# Autodesk Inventor assembly: RealSense
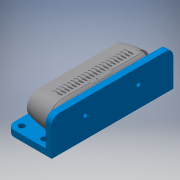
[picture p0: Inventor's stored thumbnail of the model, 180x180]
Saved by Autodesk Inventor 2019 (Build 230136000, 136)
## iProperties
Created: 2020-03-14
Part Number: RealSense
Document SubType Name: Assembly
Designer: james
Author: james
## Documents named in this file (3)
- F:\JimsRobot\FIRSTRobots\Design\Library\Jims\RealSense.iam
- F:\JimsRobot\FIRSTRobots\Design\Library\Jims\Realsense.ipt
- F:\JimsRobot\FIRSTRobots\Design\Library\Intel\000_TA_DS5_DEV_KIT_AWG_RGB_ASM__ASM.iam
## Components (2 placed, 2 different names)
1. Realsense:1 — Mate:1, Mate:2
2. 000_TA_DS5_DEV_KIT_AWG_RGB_ASM__ASM:1 [sub-assembly] — Mate:1, Mate:2
## Relationships (2: Mate 2)
- Mate:1: Realsense:1 ↔ 000_TA_DS5_DEV_KIT_AWG_RGB_ASM__ASM:1
- Mate:2: Realsense:1 ↔ 000_TA_DS5_DEV_KIT_AWG_RGB_ASM__ASM:1
